# Autodesk Inventor assembly: Link_03_Assembly
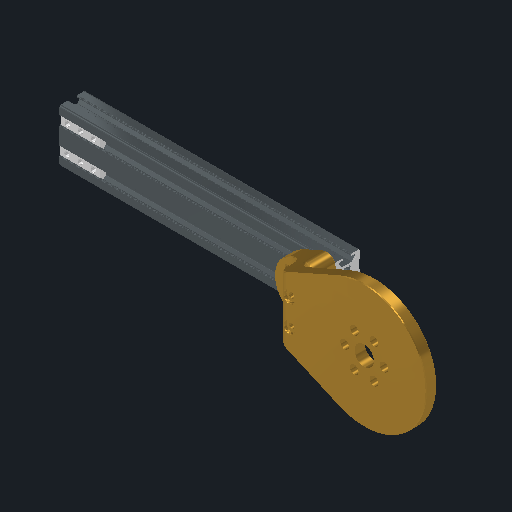
[picture p0: Inventor's stored thumbnail of the model, 512x512]
Saved by Autodesk Inventor 2026 (Build 300175000, 175)
## iProperties
Created: 2025-11-30
Part Number: Link_03_Assembly
Document SubType Name: Assembly
Designer: pochi
Mass: 279.494 g
Surface Area: 1030.35 cm^2
Volume: 154.414 cm^3
Density: 1.81004 g/cm^3
Author: pochi
## Documents named in this file (3)
- D:\POLIMI\3RD SEMESTER\Industrial Robotics\Project\Mine\Link_03_Assembly.iam
- D:\POLIMI\3RD SEMESTER\Industrial Robotics\Project\Mine\Link_03.ipt
- D:\POLIMI\3RD SEMESTER\Industrial Robotics\Project\Mine\RotationalConector_20x40.ipt
## Components (2 placed, 2 different names)
1. Link_03:1 — Mate:1, Mate:2, Mate:3
2. RotationalConector_20x40:1 — Mate:1, Mate:2, Mate:3
## Relationships (3: Mate 3)
- Mate:1: Link_03:1 ↔ RotationalConector_20x40:1
- Mate:2: Link_03:1 ↔ RotationalConector_20x40:1
- Mate:3: Link_03:1 ↔ RotationalConector_20x40:1
